# Autodesk Inventor assembly: EL2-.300
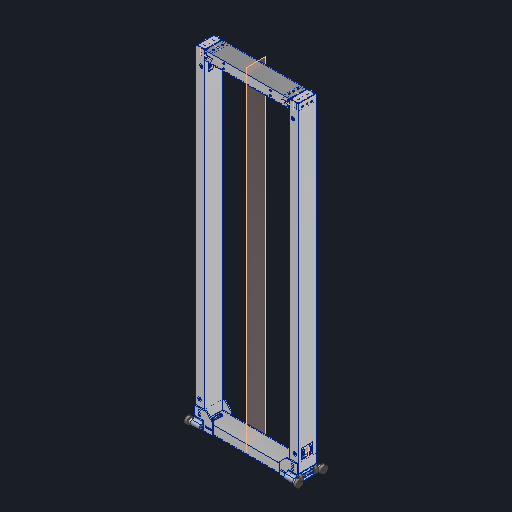
[picture p0: Inventor's stored thumbnail of the model, 512x512]
Saved by Autodesk Inventor 2023.4 (Build 274418000, 418)
## iProperties
Created: 2025-01-11
Part Number: EL2-.300
Document SubType Name: Assembly
Designer: mavericks
Author: mavericks
## Documents named in this file (8)
- C:\Users\brand\OneDrive\Documents\GitHub\robotics 23\2025-ReefScape---CAD\Elevator\EL2\EL2-.300.iam
- C:\Users\brand\OneDrive\Documents\GitHub\robotics 23\2025-ReefScape---CAD\Elevator\EL2\EL2-004.ipt
- C:\Users\brand\OneDrive\Documents\GitHub\robotics 23\2025-ReefScape---CAD\COMMON PARTS\WCP Elevator parts\WCP-0199\WCP-0199.iam
- C:\Users\brand\OneDrive\Documents\GitHub\robotics 23\2025-ReefScape---CAD\Elevator\EL2\EL2-006.ipt
- C:\Users\brand\OneDrive\Documents\GitHub\robotics 23\2025-ReefScape---CAD\Elevator\EL2\EL2-005.ipt
- C:\Users\brand\OneDrive\Documents\GitHub\robotics 23\2025-ReefScape---CAD\Elevator\EL2\EL2-400.iam
- C:\Users\brand\OneDrive\Documents\GitHub\robotics 23\2025-ReefScape---CAD\Elevator\EL2\EL2-010.ipt
- C:\Users\brand\OneDrive\Documents\GitHub\robotics 23\2025-ReefScape---CAD\Elevator\EL2\EL2-011.ipt
## Components (18 placed, 7 different names)
1. EL2-004:1 — Flush:1, Flush:2, Mate:1, Insert:3, Flush:12, Symmetry:1, Insert:4, Insert:6, Insert:8, Insert:13, Insert:14, Insert:25, Insert:29, Insert:30, Insert:32, Flush:14
2. WCP-0199:1 [sub-assembly] — Flush:1, Flush:2, Mate:1
3. EL2-011:1 — Flush:8, Insert:9, Insert:10, Insert:11, Insert:12, Insert:15, Insert:16, Insert:22, Insert:23, Insert:24, Insert:26, Insert:27, Insert:28
4. EL2-004:2 — Symmetry:1, Insert:5, Insert:7, Insert:17, Insert:18, Insert:19, Insert:20, Insert:21, Insert:31
5. WCP-0199:2 [sub-assembly] — Flush:8
6. EL2-006:3 — Flush:12, Flush:13
7. EL2-005:3
8. EL2-005:4 — Insert:3
9. EL2-400:1 [sub-assembly] — Insert:5
10. EL2-400:2 [sub-assembly] — Insert:4
11. EL2-400:3 [sub-assembly] — Insert:6
12. EL2-400:4 [sub-assembly] — Insert:7
13. EL2-010:1 — Insert:8, Insert:9, Insert:11, Insert:12, Insert:13, Insert:14
14. EL2-010:2 — Insert:10, Insert:15, Insert:16, Insert:17, Insert:18
15. EL2-010:3 — Insert:25, Insert:26, Insert:27, Insert:28, Insert:29, Insert:30
16. EL2-010:4 — Insert:19, Insert:20, Insert:21, Insert:22, Insert:23, Insert:24
17. EL2-005:5 — Flush:13, Insert:31
18. EL2-005:6 — Insert:32, Flush:14
## Relationships (47: Insert 30, Flush 11, Mate 5, Symmetry 1)
- Flush:1: EL2-004:1 ↔ WCP-0199:1
- Flush:2: EL2-004:1 ↔ WCP-0199:1
- Mate:1: EL2-004:1 ↔ WCP-0199:1
- [Flush]: EL2-004:2 ↔ WCP-0199:2
- [Flush]: EL2-004:2 ↔ WCP-0199:2
- [Mate]: EL2-004:2 ↔ WCP-0199:2
- Flush:8: EL2-011:1 ↔ WCP-0199:2
- [Flush]: EL2-006:3 ↔ EL2-005:3
- [Flush]: EL2-006:3 ↔ EL2-005:3
- [Mate]: EL2-006:3 ↔ EL2-005:3
- [Mate]: EL2-006:3 ↔ EL2-005:4
- [Mate]: EL2-006:3 ↔ EL2-005:4
- [Flush]: EL2-006:3 ↔ EL2-005:4
- Insert:3: EL2-004:1 ↔ EL2-005:4
- Flush:12: EL2-004:1 ↔ EL2-006:3
- Symmetry:1: EL2-004:1 ↔ EL2-004:2
- Insert:4: EL2-004:1 ↔ EL2-400:2
- Insert:5: EL2-004:2 ↔ EL2-400:1
- Insert:6: EL2-004:1 ↔ EL2-400:3
- Insert:7: EL2-004:2 ↔ EL2-400:4
- Insert:8: EL2-004:1 ↔ EL2-010:1
- Insert:9: EL2-011:1 ↔ EL2-010:1
- Insert:10: EL2-011:1 ↔ EL2-010:2
- Insert:11: EL2-011:1 ↔ EL2-010:1
- Insert:12: EL2-011:1 ↔ EL2-010:1
- Insert:13: EL2-004:1 ↔ EL2-010:1
- Insert:14: EL2-004:1 ↔ EL2-010:1
- Insert:15: EL2-011:1 ↔ EL2-010:2
- Insert:16: EL2-011:1 ↔ EL2-010:2
- Insert:17: EL2-004:2 ↔ EL2-010:2
- Insert:18: EL2-004:2 ↔ EL2-010:2
- Insert:19: EL2-004:2 ↔ EL2-010:4
- Insert:20: EL2-004:2 ↔ EL2-010:4
- Insert:21: EL2-004:2 ↔ EL2-010:4
- Insert:22: EL2-011:1 ↔ EL2-010:4
- Insert:23: EL2-011:1 ↔ EL2-010:4
- Insert:24: EL2-011:1 ↔ EL2-010:4
- Insert:25: EL2-004:1 ↔ EL2-010:3
- Insert:26: EL2-011:1 ↔ EL2-010:3
- Insert:27: EL2-011:1 ↔ EL2-010:3
- Insert:28: EL2-011:1 ↔ EL2-010:3
- Insert:29: EL2-004:1 ↔ EL2-010:3
- Insert:30: EL2-004:1 ↔ EL2-010:3
- Flush:13: EL2-006:3 ↔ EL2-005:5
- Insert:31: EL2-004:2 ↔ EL2-005:5
- Insert:32: EL2-004:1 ↔ EL2-005:6
- Flush:14: EL2-004:1 ↔ EL2-005:6
## Named parameters: d11_d0 = 0 mm, d12_d1 = 0 mm, d13_d2 = 0 mm, d16_d3 = 0 mm, d17_d4 = 0 mm, d18_d5 = 0 mm, d19_d6 = 0 mm, d20_d7 = 0 mm, d21_d8 = 0 mm
